# Autodesk Inventor assembly: Subframe V1
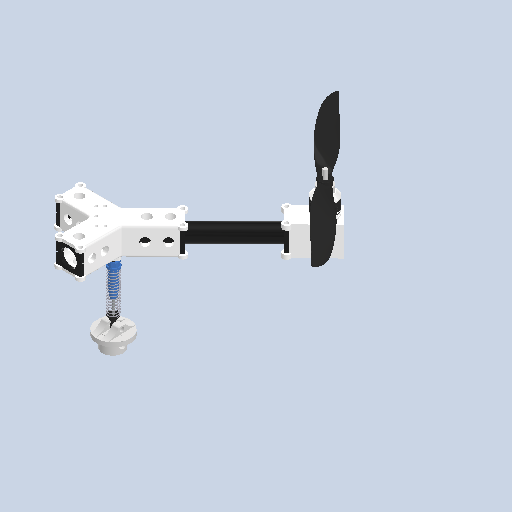
[picture p0: Inventor's stored thumbnail of the model, 512x512]
Saved by Autodesk Inventor 2022 (Build 260153000, 153)
## iProperties
Created: 2022-02-05
Part Number: Subframe V1
Document SubType Name: Assembly
Designer: ultra
Author: ultra
## Documents named in this file (9)
- C:\Users\ultra\Desktop\Github\RASA-Drone\CAD Files\Drone\Subframe V1.iam
- C:\Users\ultra\Desktop\Github\RASA-Drone\CAD Files\Drone\Tube.ipt
- C:\Users\ultra\Desktop\Github\RASA-Drone\CAD Files\Drone\TubeClamp.ipt
- C:\Users\ultra\Desktop\Github\RASA-Drone\CAD Files\Drone\BracketV3.ipt
- C:\Users\ultra\Desktop\Github\RASA-Drone\CAD Files\Drone\MotorAssembly.iam
- C:\Users\ultra\Desktop\Github\RASA-Drone\CAD Files\Drone\aeronaut_cam_carbon_light_13x5.ipt
- C:\Users\ultra\Desktop\Github\RASA-Drone\CAD Files\Drone\6633 100mm Shock absorber.ipt
- C:\Users\ultra\Desktop\Github\RASA-Drone\CAD Files\Drone\Foot.ipt
- C:\Users\ultra\Desktop\Github\RASA-Drone\CAD Files\Drone\TubeMount.ipt
## Components (13 placed, 8 different names)
1. Tube:2 — Insert:4, Insert:5
2. TubeClamp:1 — Flush:5
3. TubeClamp:2 — Flush:5
4. TubeClamp:3 — Flush:6
5. TubeClamp:4 — Flush:6
6. TubeClamp:5 — Angle:1
7. TubeClamp:6
8. BracketV3:1 — Angle:1, Insert:4, Angle:2, Insert:7
9. MotorAssembly:1 [sub-assembly] — Insert:5, Angle:2, Insert:6
10. aeronaut_cam_carbon_light_13x5:1 — Insert:6
11. 6633 100mm Shock absorber:1 — Insert:7, Insert:8, Insert:9
12. Foot:1 — Insert:8
13. TubeMount:1 — Insert:9
## Relationships (13: Insert 6, Flush 5, Angle 2)
- [Flush]: TubeClamp:1 ↔ TubeClamp:2
- [Flush]: TubeClamp:3 ↔ TubeClamp:4
- [Flush]: TubeClamp:5 ↔ TubeClamp:6
- Angle:1 (0 deg): TubeClamp:5 ↔ BracketV3:1
- Flush:5: TubeClamp:1 ↔ TubeClamp:2
- Flush:6: TubeClamp:3 ↔ TubeClamp:4
- Insert:4: Tube:2 ↔ BracketV3:1
- Insert:5: Tube:2 ↔ MotorAssembly:1
- Angle:2 (0 deg): BracketV3:1 ↔ MotorAssembly:1
- Insert:6: MotorAssembly:1 ↔ aeronaut_cam_carbon_light_13x5:1
- Insert:7: BracketV3:1 ↔ 6633 100mm Shock absorber:1
- Insert:8 (1.524 mm): 6633 100mm Shock absorber:1 ↔ Foot:1
- Insert:9: 6633 100mm Shock absorber:1 ↔ TubeMount:1
## Named parameters: d39_d38 = 0 mm, d43_d39_d38 = 0 mm
